# Autodesk Inventor assembly: undergndPipe
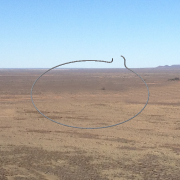
[picture p0: Inventor's stored thumbnail of the model, 180x180]
Saved by Autodesk Inventor 2014 SP1 (Build 180222100, 222)
## iProperties
Created: 2014-03-12
Part Number: undergndPipe
Document SubType Name: Assembly
Designer: Dave
Author: Dave
## Documents named in this file (3)
- C:\Users\Dave\Desktop\hera-cad\Node\undergndPipe.iam
- C:\Users\Dave\Desktop\hera-cad\Node\airgnd_exchange.ipt
- C:\Users\Dave\Desktop\hera-cad\Node\sweep.ipt
## Components (4 placed, 2 different names)
1. airgnd_exchange:1 — Insert:1, Insert:3
2. sweep:1 — Insert:1
3. sweep:2 — Insert:2
4. sweep:3 — Insert:2, Insert:3
## Relationships (3: Insert 3)
- Insert:1: airgnd_exchange:1 ↔ sweep:1
- Insert:2: sweep:2 ↔ sweep:3
- Insert:3: airgnd_exchange:1 ↔ sweep:3
